# Autodesk Inventor assembly: 73. Вал вторичный в сборе
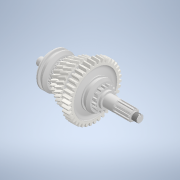
[picture p0: Inventor's stored thumbnail of the model, 180x180]
Saved by Autodesk Inventor 2021 (Build 250183000, 183)
## iProperties
Created: 2021-04-06
Part Number: 73. Вал вторичный в сборе
Document SubType Name: Assembly
Designer: Данил
Author: Данил
## Documents named in this file (12)
- C:\Users\Данил\Desktop\Коробка передач\Детали\73. Вал вторичный в сборе.iam
- C:\Users\Данил\Desktop\Коробка передач\Детали\70. Вал вторичный.ipt
- C:\Users\Данил\Desktop\Коробка передач\Детали\78. Сухарь синхронизатора.ipt
- C:\Users\Данил\Desktop\Коробка передач\Детали\69. Гайка стопорная.ipt
- C:\Users\Данил\Desktop\Коробка передач\Детали\69. Пружина синхронизатора (нагрузка).ipt
- C:\Users\Данил\Desktop\Коробка передач\Детали\74. Комплект муфты со ступицей.iam
- C:\Users\Данил\Desktop\Коробка передач\Детали\74. Втулка распорная.ipt
- C:\Users\Данил\Desktop\Коробка передач\Детали\74. Комплект шестерни с кольцом после притирки.iam
- C:\Users\Данил\Desktop\Коробка передач\Детали\69. Шайба упорная.ipt
- C:\Users\Данил\Desktop\Коробка передач\Детали\71. Шестерня первой передачи.iam
- C:\Users\Данил\Desktop\Коробка передач\Детали\68. Стопор втулки.ipt
- C:\Users\Данил\Desktop\Коробка передач\Детали\72. Шестерня второй передачи в сборе.iam
## Components (14 placed, 11 different names)
1. 70. Вал вторичный:1 — Совмещение:1, Заподлицо:2, Совмещение:4, Заподлицо:3, Совмещение:5, Совмещение:6, Совмещение:9, Заподлицо:6, Совмещение:10, Совмещение:11, Совмещение:12, Совмещение:14
2. 69. Гайка стопорная:1 — Совмещение:4, Заподлицо:3
3. 69. Пружина синхронизатора (нагрузка):1 — Совмещение:6, Совмещение:7, Заподлицо:4
4. 69. Пружина синхронизатора (нагрузка):2 — Совмещение:5, Совмещение:8, Заподлицо:5
5. 74. Комплект муфты со ступицей:1 [sub-assembly] — Совмещение:1, Совмещение:2, Совмещение:3, Заподлицо:1, Заподлицо:2, Совмещение:7, Совмещение:8, Совмещение:16
6. 74. Втулка распорная:1 — Совмещение:14, Совмещение:15, Касательность:1, Совмещение:16, Совмещение:17
7. 74. Комплект шестерни с кольцом после притирки:1 [sub-assembly] — Совмещение:17, Совмещение:18
8. 69. Шайба упорная:1 — Совмещение:12, Совмещение:13, Совмещение:18
9. 71. Шестерня первой передачи:1 [sub-assembly] — Совмещение:9, Заподлицо:6
10. 68. Стопор втулки:1 — Совмещение:15, Касательность:1
11. 72. Шестерня второй передачи в сборе:1 [sub-assembly] — Совмещение:10, Совмещение:11, Совмещение:13
12. 78. Сухарь синхронизатора:3 — Совмещение:2, Совмещение:3, Заподлицо:1, Заподлицо:4
13. 78. Сухарь синхронизатора:4 — Заподлицо:5
14. 78. Сухарь синхронизатора:5
## Component patterns: (3 elements, first: 78. Сухарь синхронизатора:3)
## Relationships (25: Mate 18, Flush 6, Tangent 1)
- Совмещение:1 [Mate]: 70. Вал вторичный:1 ↔ 74. Комплект муфты со ступицей:1
- Совмещение:2 [Mate]: 74. Комплект муфты со ступицей:1 ↔ 78. Сухарь синхронизатора:3
- Совмещение:3 [Mate]: 74. Комплект муфты со ступицей:1 ↔ 78. Сухарь синхронизатора:3
- Заподлицо:1 [Flush] (2.7 mm): 74. Комплект муфты со ступицей:1 ↔ 78. Сухарь синхронизатора:3
- Заподлицо:2 [Flush]: 70. Вал вторичный:1 ↔ 74. Комплект муфты со ступицей:1
- Совмещение:4 [Mate]: 70. Вал вторичный:1 ↔ 69. Гайка стопорная:1
- Заподлицо:3 [Flush]: 70. Вал вторичный:1 ↔ 69. Гайка стопорная:1
- Совмещение:5 [Mate]: 70. Вал вторичный:1 ↔ 69. Пружина синхронизатора (нагрузка):2
- Совмещение:6 [Mate]: 70. Вал вторичный:1 ↔ 69. Пружина синхронизатора (нагрузка):1
- Совмещение:7 [Mate] (1 mm): 69. Пружина синхронизатора (нагрузка):1 ↔ 74. Комплект муфты со ступицей:1
- Заподлицо:4 [Flush]: 69. Пружина синхронизатора (нагрузка):1 ↔ 78. Сухарь синхронизатора:3
- Совмещение:8 [Mate] (1 mm): 69. Пружина синхронизатора (нагрузка):2 ↔ 74. Комплект муфты со ступицей:1
- Заподлицо:5 [Flush]: 69. Пружина синхронизатора (нагрузка):2 ↔ 78. Сухарь синхронизатора:4
- Совмещение:9 [Mate]: 70. Вал вторичный:1 ↔ 71. Шестерня первой передачи:1
- Заподлицо:6 [Flush] (9.75 mm): 70. Вал вторичный:1 ↔ 71. Шестерня первой передачи:1
- Совмещение:10 [Mate]: 70. Вал вторичный:1 ↔ 72. Шестерня второй передачи в сборе:1
- Совмещение:11 [Mate]: 70. Вал вторичный:1 ↔ 72. Шестерня второй передачи в сборе:1
- Совмещение:12 [Mate]: 70. Вал вторичный:1 ↔ 69. Шайба упорная:1
- Совмещение:13 [Mate]: 69. Шайба упорная:1 ↔ 72. Шестерня второй передачи в сборе:1
- Совмещение:14 [Mate]: 70. Вал вторичный:1 ↔ 74. Втулка распорная:1
- Совмещение:15 [Mate]: 74. Втулка распорная:1 ↔ 68. Стопор втулки:1
- Касательность:1 [Tangent]: 74. Втулка распорная:1 ↔ 68. Стопор втулки:1
- Совмещение:16 [Mate]: 74. Комплект муфты со ступицей:1 ↔ 74. Втулка распорная:1
- Совмещение:17 [Mate]: 74. Втулка распорная:1 ↔ 74. Комплект шестерни с кольцом после притирки:1
- Совмещение:18 [Mate]: 74. Комплект шестерни с кольцом после притирки:1 ↔ 69. Шайба упорная:1
